# Autodesk Inventor assembly: inslide
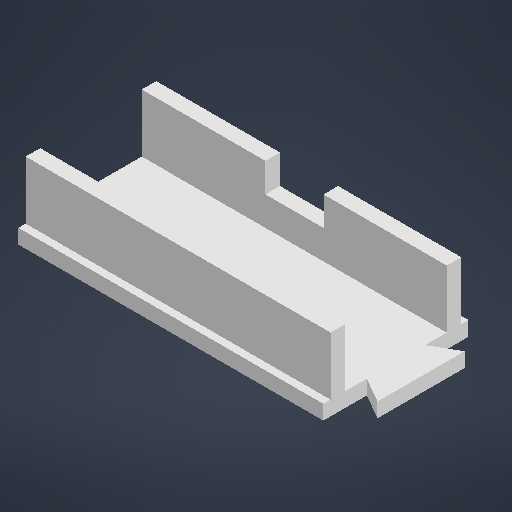
[picture p0: Inventor's stored thumbnail of the model, 512x512]
Saved by Autodesk Inventor 2026.2 (Build 302298000, 298)
## iProperties
Created: 2026-04-17
Part Number: inslide
Document SubType Name: Assembly
Designer: danda
Author: danda
## Documents named in this file (4)
- C:\Users\danda\BOM-project\Project\CAD\sorting\inslide\inslide.iam
- C:\Users\danda\BOM-project\Project\CAD\sorting\inslide\inslide2.ipt
- C:\Users\danda\BOM-project\Project\CAD\sorting\inslide\inslide1.ipt
- C:\Users\danda\BOM-project\Project\CAD\sorting\inslide\inslide3.ipt
## Components (3 placed, 3 different names)
1. inslide2:1 — Mate:1, Mate:3, Mate:4
2. inslide1:1 — Mate:1, Mate:3, Mate:4, Mate:5, Mate:6, Flush:1
3. inslide3:1 — Mate:5, Mate:6, Flush:1
## Relationships (6: Mate 5, Flush 1)
- Mate:1: inslide2:1 ↔ inslide1:1
- Mate:3: inslide2:1 ↔ inslide1:1
- Mate:4: inslide2:1 ↔ inslide1:1
- Mate:5: inslide1:1 ↔ inslide3:1
- Mate:6: inslide1:1 ↔ inslide3:1
- Flush:1: inslide1:1 ↔ inslide3:1
